(part 1 of 3)
# Autodesk Inventor assembly: COMPONENTS
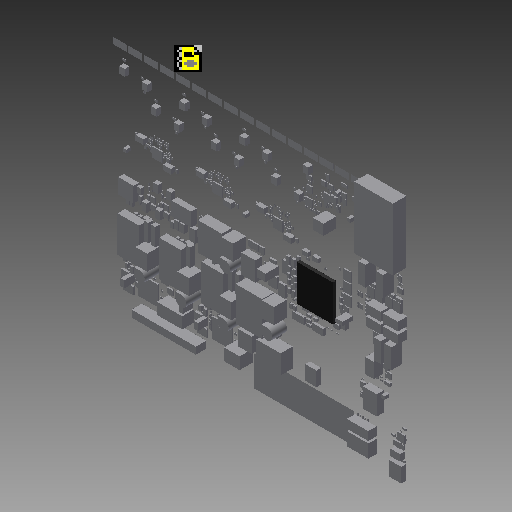
[picture p0: Inventor's stored thumbnail of the model, 512x512]
Saved by Autodesk Inventor 2017 (Build 210142000, 142)
## iProperties
Created: 2016-03-07
Part Number: COMPONENTS
Document SubType Name: Assembly
Designer: rtreacy
Author: rtreacy
## Documents named in this file (794)
- C:\Users\Zara\Documents\hera-cad\Node\SNAP_V2\Workspaces\Workspace\drawings\SNAP Ver2 pack-n-go\Workgroups\NotInProject\COMPONENTS.iam
- C:\Users\Zara\Documents\hera-cad\Node\SNAP_V2\Workspaces\Workspace\drawings\SNAP Ver2 pack-n-go\Workgroups\NotInProject\INDC1005X55L_L30.ipt
- C:\Users\Zara\Documents\hera-cad\Node\SNAP_V2\Workspaces\Workspace\drawings\SNAP Ver2 pack-n-go\Workgroups\NotInProject\INDC1005X55L_L31.ipt
- C:\Users\Zara\Documents\hera-cad\Node\SNAP_V2\Workspaces\Workspace\drawings\SNAP Ver2 pack-n-go\Workgroups\NotInProject\NRAO-LOGO_NOREFDES.ipt
- C:\Users\Zara\Documents\hera-cad\Node\SNAP_V2\Workspaces\Workspace\drawings\SNAP Ver2 pack-n-go\Workgroups\NotInProject\MOLEX_SD-74754-0220_M23.ipt
- C:\Users\Zara\Documents\hera-cad\Node\SNAP_V2\Workspaces\Workspace\drawings\SNAP Ver2 pack-n-go\Workgroups\NotInProject\SHDRRA14W55P200_7X2_1665X100-1_J11.ipt
- C:\Users\Zara\Documents\hera-cad\Node\SNAP_V2\Workspaces\Workspace\drawings\SNAP Ver2 pack-n-go\Workgroups\NotInProject\SHDRV14W55P200_7X2_1665X630H-1_J3.ipt
- C:\Users\Zara\Documents\hera-cad\Node\SNAP_V2\Workspaces\Workspace\drawings\SNAP Ver2 pack-n-go\Workgroups\NotInProject\TE_CONN_6367550-5_P3.ipt
- C:\Users\Zara\Documents\hera-cad\Node\SNAP_V2\Workspaces\Workspace\drawings\SNAP Ver2 pack-n-go\Workgroups\NotInProject\TO170P1430X470-6N-ALT1_U18.ipt
- C:\Users\Zara\Documents\hera-cad\Node\SNAP_V2\Workspaces\Workspace\drawings\SNAP Ver2 pack-n-go\Workgroups\NotInProject\SMA_END_LAUNCH_SMATP1.ipt
- C:\Users\Zara\Documents\hera-cad\Node\SNAP_V2\Workspaces\Workspace\drawings\SNAP Ver2 pack-n-go\Workgroups\NotInProject\SMA_END_LAUNCH_SMATP2.ipt
- C:\Users\Zara\Documents\hera-cad\Node\SNAP_V2\Workspaces\Workspace\drawings\SNAP Ver2 pack-n-go\Workgroups\NotInProject\SMA_END_LAUNCH_SMATP3.ipt
- C:\Users\Zara\Documents\hera-cad\Node\SNAP_V2\Workspaces\Workspace\drawings\SNAP Ver2 pack-n-go\Workgroups\NotInProject\SMA_END_LAUNCH_SMATP4.ipt
- C:\Users\Zara\Documents\hera-cad\Node\SNAP_V2\Workspaces\Workspace\drawings\SNAP Ver2 pack-n-go\Workgroups\NotInProject\SMA_END_LAUNCH_SMATP5.ipt
- C:\Users\Zara\Documents\hera-cad\Node\SNAP_V2\Workspaces\Workspace\drawings\SNAP Ver2 pack-n-go\Workgroups\NotInProject\SMA_END_LAUNCH_SMATP6.ipt
- C:\Users\Zara\Documents\hera-cad\Node\SNAP_V2\Workspaces\Workspace\drawings\SNAP Ver2 pack-n-go\Workgroups\NotInProject\SMA_END_LAUNCH_SMATP7.ipt
- C:\Users\Zara\Documents\hera-cad\Node\SNAP_V2\Workspaces\Workspace\drawings\SNAP Ver2 pack-n-go\Workgroups\NotInProject\SMA_END_LAUNCH_SMATP8.ipt
- C:\Users\Zara\Documents\hera-cad\Node\SNAP_V2\Workspaces\Workspace\drawings\SNAP Ver2 pack-n-go\Workgroups\NotInProject\SMA_END_LAUNCH_SMATP9.ipt
- C:\Users\Zara\Documents\hera-cad\Node\SNAP_V2\Workspaces\Workspace\drawings\SNAP Ver2 pack-n-go\Workgroups\NotInProject\SMA_END_LAUNCH_SMATP10.ipt
- C:\Users\Zara\Documents\hera-cad\Node\SNAP_V2\Workspaces\Workspace\drawings\SNAP Ver2 pack-n-go\Workgroups\NotInProject\SMA_END_LAUNCH_SMATP11.ipt
- C:\Users\Zara\Documents\hera-cad\Node\SNAP_V2\Workspaces\Workspace\drawings\SNAP Ver2 pack-n-go\Workgroups\NotInProject\SMA_END_LAUNCH_SMATP12.ipt
- C:\Users\Zara\Documents\hera-cad\Node\SNAP_V2\Workspaces\Workspace\drawings\SNAP Ver2 pack-n-go\Workgroups\NotInProject\SMA_END_LAUNCH_SMATP13.ipt
- C:\Users\Zara\Documents\hera-cad\Node\SNAP_V2\Workspaces\Workspace\drawings\SNAP Ver2 pack-n-go\Workgroups\NotInProject\SMA_END_LAUNCH_SMATP14.ipt
- C:\Users\Zara\Documents\hera-cad\Node\SNAP_V2\Workspaces\Workspace\drawings\SNAP Ver2 pack-n-go\Workgroups\NotInProject\SMA_END_LAUNCH_SMATP15.ipt
- C:\Users\Zara\Documents\hera-cad\Node\SNAP_V2\Workspaces\Workspace\drawings\SNAP Ver2 pack-n-go\Workgroups\NotInProject\SMA_END_LAUNCH_SMATP16.ipt
- C:\Users\Zara\Documents\hera-cad\Node\SNAP_V2\Workspaces\Workspace\drawings\SNAP Ver2 pack-n-go\Workgroups\NotInProject\HDRV254W64P254R1L508T254H838_JP3.ipt
- C:\Users\Zara\Documents\hera-cad\Node\SNAP_V2\Workspaces\Workspace\drawings\SNAP Ver2 pack-n-go\Workgroups\NotInProject\HDRV254W64P254R1L508T254H838_JP2.ipt
- C:\Users\Zara\Documents\hera-cad\Node\SNAP_V2\Workspaces\Workspace\drawings\SNAP Ver2 pack-n-go\Workgroups\NotInProject\HDRV254W64P254R1L508T254H838_JP1.ipt
- C:\Users\Zara\Documents\hera-cad\Node\SNAP_V2\Workspaces\Workspace\drawings\SNAP Ver2 pack-n-go\Workgroups\NotInProject\HDRV254W64P254R1L508T254H838_JP4.ipt
- C:\Users\Zara\Documents\hera-cad\Node\SNAP_V2\Workspaces\Workspace\drawings\SNAP Ver2 pack-n-go\Workgroups\NotInProject\HDRV6X2_J9.ipt
- C:\Users\Zara\Documents\hera-cad\Node\SNAP_V2\Workspaces\Workspace\drawings\SNAP Ver2 pack-n-go\Workgroups\NotInProject\HDRV6X2_J7.ipt
- C:\Users\Zara\Documents\hera-cad\Node\SNAP_V2\Workspaces\Workspace\drawings\SNAP Ver2 pack-n-go\Workgroups\NotInProject\HDRV6X2_J5.ipt
- C:\Users\Zara\Documents\hera-cad\Node\SNAP_V2\Workspaces\Workspace\drawings\SNAP Ver2 pack-n-go\Workgroups\NotInProject\HDRV6X2_J6.ipt
- C:\Users\Zara\Documents\hera-cad\Node\SNAP_V2\Workspaces\Workspace\drawings\SNAP Ver2 pack-n-go\Workgroups\NotInProject\HDRV2X20_PI2.ipt
- C:\Users\Zara\Documents\hera-cad\Node\SNAP_V2\Workspaces\Workspace\drawings\SNAP Ver2 pack-n-go\Workgroups\NotInProject\CAPPRD350W60D820H1170P_C259.ipt
- C:\Users\Zara\Documents\hera-cad\Node\SNAP_V2\Workspaces\Workspace\drawings\SNAP Ver2 pack-n-go\Workgroups\NotInProject\CAPPRD350W60D820H1170P_C250.ipt
- C:\Users\Zara\Documents\hera-cad\Node\SNAP_V2\Workspaces\Workspace\drawings\SNAP Ver2 pack-n-go\Workgroups\NotInProject\CAPPRD350W60D820H1170P_C241.ipt
- C:\Users\Zara\Documents\hera-cad\Node\SNAP_V2\Workspaces\Workspace\drawings\SNAP Ver2 pack-n-go\Workgroups\NotInProject\CAPPRD350W60D820H1170P_C234.ipt
- C:\Users\Zara\Documents\hera-cad\Node\SNAP_V2\Workspaces\Workspace\drawings\SNAP Ver2 pack-n-go\Workgroups\NotInProject\CAPPRD350W60D820H1170P_C227.ipt
- C:\Users\Zara\Documents\hera-cad\Node\SNAP_V2\Workspaces\Workspace\drawings\SNAP Ver2 pack-n-go\Workgroups\NotInProject\QFN50P500X500X100-28N_U29.ipt
- C:\Users\Zara\Documents\hera-cad\Node\SNAP_V2\Workspaces\Workspace\drawings\SNAP Ver2 pack-n-go\Workgroups\NotInProject\FID100X125_NOREFDES.ipt
- C:\Users\Zara\Documents\hera-cad\Node\SNAP_V2\Workspaces\Workspace\drawings\SNAP Ver2 pack-n-go\Workgroups\NotInProject\DIOAD1365W102L865D350B_D4.ipt
- C:\Users\Zara\Documents\hera-cad\Node\SNAP_V2\Workspaces\Workspace\drawings\SNAP Ver2 pack-n-go\Workgroups\NotInProject\DIOAD1365W102L865D350B_D5.ipt
- C:\Users\Zara\Documents\hera-cad\Node\SNAP_V2\Workspaces\Workspace\drawings\SNAP Ver2 pack-n-go\Workgroups\NotInProject\DIOAD1365W102L865D350B_D6.ipt
- C:\Users\Zara\Documents\hera-cad\Node\SNAP_V2\Workspaces\Workspace\drawings\SNAP Ver2 pack-n-go\Workgroups\NotInProject\DIOAD1365W102L865D350B_D7.ipt
- C:\Users\Zara\Documents\hera-cad\Node\SNAP_V2\Workspaces\Workspace\drawings\SNAP Ver2 pack-n-go\Workgroups\NotInProject\DIOAD1365W102L865D350B_D8.ipt
- C:\Users\Zara\Documents\hera-cad\Node\SNAP_V2\Workspaces\Workspace\drawings\SNAP Ver2 pack-n-go\Workgroups\NotInProject\BGA676C100P26X26_2700X2700X260_U25.ipt
- C:\Users\Zara\Documents\hera-cad\Node\SNAP_V2\Workspaces\Workspace\drawings\SNAP Ver2 pack-n-go\Workgroups\NotInProject\EMERSON_RFCONN_SMA-V_TP2.ipt
- C:\Users\Zara\Documents\hera-cad\Node\SNAP_V2\Workspaces\Workspace\drawings\SNAP Ver2 pack-n-go\Workgroups\NotInProject\FIL_BNX01X_U24.ipt
- C:\Users\Zara\Documents\hera-cad\Node\SNAP_V2\Workspaces\Workspace\drawings\SNAP Ver2 pack-n-go\Workgroups\NotInProject\MOLEX_744410010_P2.ipt
- C:\Users\Zara\Documents\hera-cad\Node\SNAP_V2\Workspaces\Workspace\drawings\SNAP Ver2 pack-n-go\Workgroups\NotInProject\MOLEX_744410010_P1.ipt
- C:\Users\Zara\Documents\hera-cad\Node\SNAP_V2\Workspaces\Workspace\drawings\SNAP Ver2 pack-n-go\Workgroups\NotInProject\SOT89_Q5.ipt
- C:\Users\Zara\Documents\hera-cad\Node\SNAP_V2\Workspaces\Workspace\drawings\SNAP Ver2 pack-n-go\Workgroups\NotInProject\SOT89_Q6.ipt
- C:\Users\Zara\Documents\hera-cad\Node\SNAP_V2\Workspaces\Workspace\drawings\SNAP Ver2 pack-n-go\Workgroups\NotInProject\QFN80P1000X1000X440-42T320X130X2N-ALT1_U20.ipt
- C:\Users\Zara\Documents\hera-cad\Node\SNAP_V2\Workspaces\Workspace\drawings\SNAP Ver2 pack-n-go\Workgroups\NotInProject\HDR_1X2_LOCK_MOLEX_J61.ipt
- C:\Users\Zara\Documents\hera-cad\Node\SNAP_V2\Workspaces\Workspace\drawings\SNAP Ver2 pack-n-go\Workgroups\NotInProject\DIOMELF3514_D14.ipt
- C:\Users\Zara\Documents\hera-cad\Node\SNAP_V2\Workspaces\Workspace\drawings\SNAP Ver2 pack-n-go\Workgroups\NotInProject\SOT230P700X180-4L050N_Q17.ipt
- C:\Users\Zara\Documents\hera-cad\Node\SNAP_V2\Workspaces\Workspace\drawings\SNAP Ver2 pack-n-go\Workgroups\NotInProject\QFP50P1400X1400X100-80N_U40.ipt
- C:\Users\Zara\Documents\hera-cad\Node\SNAP_V2\Workspaces\Workspace\drawings\SNAP Ver2 pack-n-go\Workgroups\NotInProject\QFP50P1400X1400X100-80N_U42.ipt
- C:\Users\Zara\Documents\hera-cad\Node\SNAP_V2\Workspaces\Workspace\drawings\SNAP Ver2 pack-n-go\Workgroups\NotInProject\QFN50P700X700X100-49T540X540L_U7.ipt
- C:\Users\Zara\Documents\hera-cad\Node\SNAP_V2\Workspaces\Workspace\drawings\SNAP Ver2 pack-n-go\Workgroups\NotInProject\QFN50P700X700X100-49T540X540L_U2.ipt
- C:\Users\Zara\Documents\hera-cad\Node\SNAP_V2\Workspaces\Workspace\drawings\SNAP Ver2 pack-n-go\Workgroups\NotInProject\QFN50P700X700X100-49T540X540L_U12.ipt
- C:\Users\Zara\Documents\hera-cad\Node\SNAP_V2\Workspaces\Workspace\drawings\SNAP Ver2 pack-n-go\Workgroups\NotInProject\QFN50P500X500X100-33T320X320L_U21.ipt
- C:\Users\Zara\Documents\hera-cad\Node\SNAP_V2\Workspaces\Workspace\drawings\SNAP Ver2 pack-n-go\Workgroups\NotInProject\QFN50P500X500X100-33T380X380L_U23.ipt
- C:\Users\Zara\Documents\hera-cad\Node\SNAP_V2\Workspaces\Workspace\drawings\SNAP Ver2 pack-n-go\Workgroups\NotInProject\QFN50P400X400X100-25T280X280L_U22.ipt
- C:\Users\Zara\Documents\hera-cad\Node\SNAP_V2\Workspaces\Workspace\drawings\SNAP Ver2 pack-n-go\Workgroups\NotInProject\DCDC-CONV_PTD08D210W-22N_U38.ipt
- C:\Users\Zara\Documents\hera-cad\Node\SNAP_V2\Workspaces\Workspace\drawings\SNAP Ver2 pack-n-go\Workgroups\NotInProject\DCDC-CONV_PTD08D210W-22N_U36.ipt
- C:\Users\Zara\Documents\hera-cad\Node\SNAP_V2\Workspaces\Workspace\drawings\SNAP Ver2 pack-n-go\Workgroups\NotInProject\DCDC-CONV_PTD08D210W-22N_U37.ipt
- C:\Users\Zara\Documents\hera-cad\Node\SNAP_V2\Workspaces\Workspace\drawings\SNAP Ver2 pack-n-go\Workgroups\NotInProject\QFN50P300X300X100-17T178X178L_U17.ipt
- C:\Users\Zara\Documents\hera-cad\Node\SNAP_V2\Workspaces\Workspace\drawings\SNAP Ver2 pack-n-go\Workgroups\NotInProject\QFN50P300X300X100-17T178X178L_U16.ipt
- C:\Users\Zara\Documents\hera-cad\Node\SNAP_V2\Workspaces\Workspace\drawings\SNAP Ver2 pack-n-go\Workgroups\NotInProject\SOP65P640X120-16N_U41.ipt
- C:\Users\Zara\Documents\hera-cad\Node\SNAP_V2\Workspaces\Workspace\drawings\SNAP Ver2 pack-n-go\Workgroups\NotInProject\SOP65P640X120-16N_U39.ipt
- C:\Users\Zara\Documents\hera-cad\Node\SNAP_V2\Workspaces\Workspace\drawings\SNAP Ver2 pack-n-go\Workgroups\NotInProject\QFN40P260X180X55-16L_U28.ipt
- C:\Users\Zara\Documents\hera-cad\Node\SNAP_V2\Workspaces\Workspace\drawings\SNAP Ver2 pack-n-go\Workgroups\NotInProject\QFN40P260X180X55-16L_U46.ipt
- C:\Users\Zara\Documents\hera-cad\Node\SNAP_V2\Workspaces\Workspace\drawings\SNAP Ver2 pack-n-go\Workgroups\NotInProject\QFN40P260X180X55-16L_U47.ipt
- C:\Users\Zara\Documents\hera-cad\Node\SNAP_V2\Workspaces\Workspace\drawings\SNAP Ver2 pack-n-go\Workgroups\NotInProject\DCDC-CONV_PTD08A020WAD-12N_U35.ipt
- C:\Users\Zara\Documents\hera-cad\Node\SNAP_V2\Workspaces\Workspace\drawings\SNAP Ver2 pack-n-go\Workgroups\NotInProject\DCDC-CONV_PTD08A010WAD-12N_U34.ipt
- C:\Users\Zara\Documents\hera-cad\Node\SNAP_V2\Workspaces\Workspace\drawings\SNAP Ver2 pack-n-go\Workgroups\NotInProject\HDRV1016W64P254R2L2032T905H900_J1.ipt
- C:\Users\Zara\Documents\hera-cad\Node\SNAP_V2\Workspaces\Workspace\drawings\SNAP Ver2 pack-n-go\Workgroups\NotInProject\SW_SDA05H1SBD_S2.ipt
- C:\Users\Zara\Documents\hera-cad\Node\SNAP_V2\Workspaces\Workspace\drawings\SNAP Ver2 pack-n-go\Workgroups\NotInProject\SW_SDA05H1SBD_S1.ipt
- C:\Users\Zara\Documents\hera-cad\Node\SNAP_V2\Workspaces\Workspace\drawings\SNAP Ver2 pack-n-go\Workgroups\NotInProject\MOLEX_548190589_J4.ipt
- C:\Users\Zara\Documents\hera-cad\Node\SNAP_V2\Workspaces\Workspace\drawings\SNAP Ver2 pack-n-go\Workgroups\NotInProject\SOP50P310X90-8N_U44.ipt
- C:\Users\Zara\Documents\hera-cad\Node\SNAP_V2\Workspaces\Workspace\drawings\SNAP Ver2 pack-n-go\Workgroups\NotInProject\SOP50P310X90-8N_U45.ipt
- C:\Users\Zara\Documents\hera-cad\Node\SNAP_V2\Workspaces\Workspace\drawings\SNAP Ver2 pack-n-go\Workgroups\NotInProject\OSC254P700X500X90-7T147X230N_U32.ipt
- C:\Users\Zara\Documents\hera-cad\Node\SNAP_V2\Workspaces\Workspace\drawings\SNAP Ver2 pack-n-go\Workgroups\NotInProject\MOLEX_39301060_J2.ipt
- C:\Users\Zara\Documents\hera-cad\Node\SNAP_V2\Workspaces\Workspace\drawings\SNAP Ver2 pack-n-go\Workgroups\NotInProject\SOT95P280X145-6N_U26.ipt
- C:\Users\Zara\Documents\hera-cad\Node\SNAP_V2\Workspaces\Workspace\drawings\SNAP Ver2 pack-n-go\Workgroups\NotInProject\OSC254P700X500X90-6N_U48.ipt
- C:\Users\Zara\Documents\hera-cad\Node\SNAP_V2\Workspaces\Workspace\drawings\SNAP Ver2 pack-n-go\Workgroups\NotInProject\OSC254P700X500X90-6N_U33.ipt
- C:\Users\Zara\Documents\hera-cad\Node\SNAP_V2\Workspaces\Workspace\drawings\SNAP Ver2 pack-n-go\Workgroups\NotInProject\XFMR_TC1-1-13MG2_T11.ipt
- C:\Users\Zara\Documents\hera-cad\Node\SNAP_V2\Workspaces\Workspace\drawings\SNAP Ver2 pack-n-go\Workgroups\NotInProject\XFMR_TC1-1-13MG2_T10.ipt
- C:\Users\Zara\Documents\hera-cad\Node\SNAP_V2\Workspaces\Workspace\drawings\SNAP Ver2 pack-n-go\Workgroups\NotInProject\XFMR_TC1-1-13MG2_T4.ipt
- C:\Users\Zara\Documents\hera-cad\Node\SNAP_V2\Workspaces\Workspace\drawings\SNAP Ver2 pack-n-go\Workgroups\NotInProject\XFMR_TC1-1-13MG2_T6.ipt
- C:\Users\Zara\Documents\hera-cad\Node\SNAP_V2\Workspaces\Workspace\drawings\SNAP Ver2 pack-n-go\Workgroups\NotInProject\XFMR_TC1-1-13MG2_T12.ipt
- C:\Users\Zara\Documents\hera-cad\Node\SNAP_V2\Workspaces\Workspace\drawings\SNAP Ver2 pack-n-go\Workgroups\NotInProject\XFMR_TC1-1-13MG2_T5.ipt
- C:\Users\Zara\Documents\hera-cad\Node\SNAP_V2\Workspaces\Workspace\drawings\SNAP Ver2 pack-n-go\Workgroups\NotInProject\XFMR_TC1-1-13MG2_T3.ipt
- C:\Users\Zara\Documents\hera-cad\Node\SNAP_V2\Workspaces\Workspace\drawings\SNAP Ver2 pack-n-go\Workgroups\NotInProject\XFMR_TC1-1-13MG2_T8.ipt
- C:\Users\Zara\Documents\hera-cad\Node\SNAP_V2\Workspaces\Workspace\drawings\SNAP Ver2 pack-n-go\Workgroups\NotInProject\XFMR_TC1-1-13MG2_T9.ipt
- C:\Users\Zara\Documents\hera-cad\Node\SNAP_V2\Workspaces\Workspace\drawings\SNAP Ver2 pack-n-go\Workgroups\NotInProject\XFMR_TC1-1-13MG2_T13.ipt
- C:\Users\Zara\Documents\hera-cad\Node\SNAP_V2\Workspaces\Workspace\drawings\SNAP Ver2 pack-n-go\Workgroups\NotInProject\XFMR_TC1-1-13MG2_T2.ipt
- C:\Users\Zara\Documents\hera-cad\Node\SNAP_V2\Workspaces\Workspace\drawings\SNAP Ver2 pack-n-go\Workgroups\NotInProject\XFMR_TC1-1-13MG2_T7.ipt
- C:\Users\Zara\Documents\hera-cad\Node\SNAP_V2\Workspaces\Workspace\drawings\SNAP Ver2 pack-n-go\Workgroups\NotInProject\XFMR_TC1-1-13MG2_T1.ipt
- C:\Users\Zara\Documents\hera-cad\Node\SNAP_V2\Workspaces\Workspace\drawings\SNAP Ver2 pack-n-go\Workgroups\NotInProject\SOT95P280X145-5N_U30.ipt
- C:\Users\Zara\Documents\hera-cad\Node\SNAP_V2\Workspaces\Workspace\drawings\SNAP Ver2 pack-n-go\Workgroups\NotInProject\SOT95P280X145-5N_U19.ipt
- C:\Users\Zara\Documents\hera-cad\Node\SNAP_V2\Workspaces\Workspace\drawings\SNAP Ver2 pack-n-go\Workgroups\NotInProject\SOT143R_X1.ipt
- C:\Users\Zara\Documents\hera-cad\Node\SNAP_V2\Workspaces\Workspace\drawings\SNAP Ver2 pack-n-go\Workgroups\NotInProject\RESCAF65P100X100X45-4N_U10.ipt
- C:\Users\Zara\Documents\hera-cad\Node\SNAP_V2\Workspaces\Workspace\drawings\SNAP Ver2 pack-n-go\Workgroups\NotInProject\RESCAF65P100X100X45-4N_U1.ipt
- C:\Users\Zara\Documents\hera-cad\Node\SNAP_V2\Workspaces\Workspace\drawings\SNAP Ver2 pack-n-go\Workgroups\NotInProject\RESCAF65P100X100X45-4N_U11.ipt
- C:\Users\Zara\Documents\hera-cad\Node\SNAP_V2\Workspaces\Workspace\drawings\SNAP Ver2 pack-n-go\Workgroups\NotInProject\RESCAF65P100X100X45-4N_U13.ipt
- C:\Users\Zara\Documents\hera-cad\Node\SNAP_V2\Workspaces\Workspace\drawings\SNAP Ver2 pack-n-go\Workgroups\NotInProject\RESCAF65P100X100X45-4N_U14.ipt
- C:\Users\Zara\Documents\hera-cad\Node\SNAP_V2\Workspaces\Workspace\drawings\SNAP Ver2 pack-n-go\Workgroups\NotInProject\RESCAF65P100X100X45-4N_U15.ipt
- C:\Users\Zara\Documents\hera-cad\Node\SNAP_V2\Workspaces\Workspace\drawings\SNAP Ver2 pack-n-go\Workgroups\NotInProject\RESCAF65P100X100X45-4N_U3.ipt
- C:\Users\Zara\Documents\hera-cad\Node\SNAP_V2\Workspaces\Workspace\drawings\SNAP Ver2 pack-n-go\Workgroups\NotInProject\RESCAF65P100X100X45-4N_U4.ipt
- C:\Users\Zara\Documents\hera-cad\Node\SNAP_V2\Workspaces\Workspace\drawings\SNAP Ver2 pack-n-go\Workgroups\NotInProject\RESCAF65P100X100X45-4N_U5.ipt
- C:\Users\Zara\Documents\hera-cad\Node\SNAP_V2\Workspaces\Workspace\drawings\SNAP Ver2 pack-n-go\Workgroups\NotInProject\RESCAF65P100X100X45-4N_U6.ipt
- C:\Users\Zara\Documents\hera-cad\Node\SNAP_V2\Workspaces\Workspace\drawings\SNAP Ver2 pack-n-go\Workgroups\NotInProject\RESCAF65P100X100X45-4N_U8.ipt
- C:\Users\Zara\Documents\hera-cad\Node\SNAP_V2\Workspaces\Workspace\drawings\SNAP Ver2 pack-n-go\Workgroups\NotInProject\RESCAF65P100X100X45-4N_U9.ipt
- C:\Users\Zara\Documents\hera-cad\Node\SNAP_V2\Workspaces\Workspace\drawings\SNAP Ver2 pack-n-go\Workgroups\NotInProject\SW_TL3301EF100QG_SW5.ipt
- C:\Users\Zara\Documents\hera-cad\Node\SNAP_V2\Workspaces\Workspace\drawings\SNAP Ver2 pack-n-go\Workgroups\NotInProject\SW_TL3301EF100QG_SW4.ipt
- C:\Users\Zara\Documents\hera-cad\Node\SNAP_V2\Workspaces\Workspace\drawings\SNAP Ver2 pack-n-go\Workgroups\NotInProject\SW_TL3301EF100QG_SW3.ipt
- C:\Users\Zara\Documents\hera-cad\Node\SNAP_V2\Workspaces\Workspace\drawings\SNAP Ver2 pack-n-go\Workgroups\NotInProject\SW_TL3301EF100QG_SW2.ipt
- C:\Users\Zara\Documents\hera-cad\Node\SNAP_V2\Workspaces\Workspace\drawings\SNAP Ver2 pack-n-go\Workgroups\NotInProject\SW_TL3301EF100QG_SW1.ipt
- C:\Users\Zara\Documents\hera-cad\Node\SNAP_V2\Workspaces\Workspace\drawings\SNAP Ver2 pack-n-go\Workgroups\NotInProject\SOT192P237X112-4L20N_D3.ipt
- C:\Users\Zara\Documents\hera-cad\Node\SNAP_V2\Workspaces\Workspace\drawings\SNAP Ver2 pack-n-go\Workgroups\NotInProject\SOT95P237X100-4_Q1.ipt
- C:\Users\Zara\Documents\hera-cad\Node\SNAP_V2\Workspaces\Workspace\drawings\SNAP Ver2 pack-n-go\Workgroups\NotInProject\SOT95P237X100-4_Q4.ipt
- C:\Users\Zara\Documents\hera-cad\Node\SNAP_V2\Workspaces\Workspace\drawings\SNAP Ver2 pack-n-go\Workgroups\NotInProject\SOT95P237X100-4_Q3.ipt
- C:\Users\Zara\Documents\hera-cad\Node\SNAP_V2\Workspaces\Workspace\drawings\SNAP Ver2 pack-n-go\Workgroups\NotInProject\SOT95P237X100-4_Q2.ipt
- C:\Users\Zara\Documents\hera-cad\Node\SNAP_V2\Workspaces\Workspace\drawings\SNAP Ver2 pack-n-go\Workgroups\NotInProject\SOT95P237X100-4_Q8.ipt
- C:\Users\Zara\Documents\hera-cad\Node\SNAP_V2\Workspaces\Workspace\drawings\SNAP Ver2 pack-n-go\Workgroups\NotInProject\SOT95P237X100-4_Q7.ipt
- C:\Users\Zara\Documents\hera-cad\Node\SNAP_V2\Workspaces\Workspace\drawings\SNAP Ver2 pack-n-go\Workgroups\NotInProject\SOT95P240X110-3L16N_U31.ipt
- C:\Users\Zara\Documents\hera-cad\Node\SNAP_V2\Workspaces\Workspace\drawings\SNAP Ver2 pack-n-go\Workgroups\NotInProject\SOT95P240X110-3L16N_D1.ipt
- C:\Users\Zara\Documents\hera-cad\Node\SNAP_V2\Workspaces\Workspace\drawings\SNAP Ver2 pack-n-go\Workgroups\NotInProject\SOT95P240X110-3L16N_D2.ipt
- C:\Users\Zara\Documents\hera-cad\Node\SNAP_V2\Workspaces\Workspace\drawings\SNAP Ver2 pack-n-go\Workgroups\NotInProject\CAPC1005X50L_C604.ipt
- C:\Users\Zara\Documents\hera-cad\Node\SNAP_V2\Workspaces\Workspace\drawings\SNAP Ver2 pack-n-go\Workgroups\NotInProject\CAPC1005X50L_C603.ipt
- C:\Users\Zara\Documents\hera-cad\Node\SNAP_V2\Workspaces\Workspace\drawings\SNAP Ver2 pack-n-go\Workgroups\NotInProject\CAPC1005X50L_C591.ipt
- C:\Users\Zara\Documents\hera-cad\Node\SNAP_V2\Workspaces\Workspace\drawings\SNAP Ver2 pack-n-go\Workgroups\NotInProject\CAPC1005X50L_C592.ipt
- C:\Users\Zara\Documents\hera-cad\Node\SNAP_V2\Workspaces\Workspace\drawings\SNAP Ver2 pack-n-go\Workgroups\NotInProject\CAPC1005X50L_C593.ipt
- C:\Users\Zara\Documents\hera-cad\Node\SNAP_V2\Workspaces\Workspace\drawings\SNAP Ver2 pack-n-go\Workgroups\NotInProject\CAPC1005X50L_C46.ipt
- C:\Users\Zara\Documents\hera-cad\Node\SNAP_V2\Workspaces\Workspace\drawings\SNAP Ver2 pack-n-go\Workgroups\NotInProject\CAPC1005X50L_C51.ipt
- C:\Users\Zara\Documents\hera-cad\Node\SNAP_V2\Workspaces\Workspace\drawings\SNAP Ver2 pack-n-go\Workgroups\NotInProject\CAPC1005X50L_C57.ipt
- C:\Users\Zara\Documents\hera-cad\Node\SNAP_V2\Workspaces\Workspace\drawings\SNAP Ver2 pack-n-go\Workgroups\NotInProject\CAPC1005X50L_C7.ipt
- C:\Users\Zara\Documents\hera-cad\Node\SNAP_V2\Workspaces\Workspace\drawings\SNAP Ver2 pack-n-go\Workgroups\NotInProject\CAPC1005X50L_C82.ipt
- C:\Users\Zara\Documents\hera-cad\Node\SNAP_V2\Workspaces\Workspace\drawings\SNAP Ver2 pack-n-go\Workgroups\NotInProject\CAPC1005X50L_C43.ipt
- C:\Users\Zara\Documents\hera-cad\Node\SNAP_V2\Workspaces\Workspace\drawings\SNAP Ver2 pack-n-go\Workgroups\NotInProject\CAPC1005X50L_C96.ipt
- C:\Users\Zara\Documents\hera-cad\Node\SNAP_V2\Workspaces\Workspace\drawings\SNAP Ver2 pack-n-go\Workgroups\NotInProject\CAPC1005X50L_C85.ipt
- C:\Users\Zara\Documents\hera-cad\Node\SNAP_V2\Workspaces\Workspace\drawings\SNAP Ver2 pack-n-go\Workgroups\NotInProject\CAPC1005X50L_C90.ipt
- C:\Users\Zara\Documents\hera-cad\Node\SNAP_V2\Workspaces\Workspace\drawings\SNAP Ver2 pack-n-go\Workgroups\NotInProject\CAPC1005X50L_C13.ipt
- C:\Users\Zara\Documents\hera-cad\Node\SNAP_V2\Workspaces\Workspace\drawings\SNAP Ver2 pack-n-go\Workgroups\NotInProject\CAPC1005X50L_C4.ipt
- C:\Users\Zara\Documents\hera-cad\Node\SNAP_V2\Workspaces\Workspace\drawings\SNAP Ver2 pack-n-go\Workgroups\NotInProject\CAPC1005X50L_C47.ipt
- C:\Users\Zara\Documents\hera-cad\Node\SNAP_V2\Workspaces\Workspace\drawings\SNAP Ver2 pack-n-go\Workgroups\NotInProject\CAPC1005X50L_C5.ipt
- C:\Users\Zara\Documents\hera-cad\Node\SNAP_V2\Workspaces\Workspace\drawings\SNAP Ver2 pack-n-go\Workgroups\NotInProject\CAPC1005X50L_C52.ipt
- C:\Users\Zara\Documents\hera-cad\Node\SNAP_V2\Workspaces\Workspace\drawings\SNAP Ver2 pack-n-go\Workgroups\NotInProject\CAPC1005X50L_C58.ipt
- C:\Users\Zara\Documents\hera-cad\Node\SNAP_V2\Workspaces\Workspace\drawings\SNAP Ver2 pack-n-go\Workgroups\NotInProject\CAPC1005X50L_C8.ipt
- C:\Users\Zara\Documents\hera-cad\Node\SNAP_V2\Workspaces\Workspace\drawings\SNAP Ver2 pack-n-go\Workgroups\NotInProject\CAPC1005X50L_C83.ipt
- C:\Users\Zara\Documents\hera-cad\Node\SNAP_V2\Workspaces\Workspace\drawings\SNAP Ver2 pack-n-go\Workgroups\NotInProject\CAPC1005X50L_C86.ipt
- C:\Users\Zara\Documents\hera-cad\Node\SNAP_V2\Workspaces\Workspace\drawings\SNAP Ver2 pack-n-go\Workgroups\NotInProject\CAPC1005X50L_C91.ipt
- C:\Users\Zara\Documents\hera-cad\Node\SNAP_V2\Workspaces\Workspace\drawings\SNAP Ver2 pack-n-go\Workgroups\NotInProject\CAPC1005X50L_C97.ipt
- C:\Users\Zara\Documents\hera-cad\Node\SNAP_V2\Workspaces\Workspace\drawings\SNAP Ver2 pack-n-go\Workgroups\NotInProject\CAPC1005X50L_C19.ipt
- C:\Users\Zara\Documents\hera-cad\Node\SNAP_V2\Workspaces\Workspace\drawings\SNAP Ver2 pack-n-go\Workgroups\NotInProject\CAPC1005X50L_C14.ipt
- C:\Users\Zara\Documents\hera-cad\Node\SNAP_V2\Workspaces\Workspace\drawings\SNAP Ver2 pack-n-go\Workgroups\NotInProject\CAPC1005X50L_C17.ipt
- C:\Users\Zara\Documents\hera-cad\Node\SNAP_V2\Workspaces\Workspace\drawings\SNAP Ver2 pack-n-go\Workgroups\NotInProject\CAPC1005X50L_C2.ipt
- C:\Users\Zara\Documents\hera-cad\Node\SNAP_V2\Workspaces\Workspace\drawings\SNAP Ver2 pack-n-go\Workgroups\NotInProject\CAPC1005X50L_C41.ipt
- C:\Users\Zara\Documents\hera-cad\Node\SNAP_V2\Workspaces\Workspace\drawings\SNAP Ver2 pack-n-go\Workgroups\NotInProject\CAPC1005X50L_C44.ipt
- C:\Users\Zara\Documents\hera-cad\Node\SNAP_V2\Workspaces\Workspace\drawings\SNAP Ver2 pack-n-go\Workgroups\NotInProject\CAPC1005X50L_C53.ipt
- C:\Users\Zara\Documents\hera-cad\Node\SNAP_V2\Workspaces\Workspace\drawings\SNAP Ver2 pack-n-go\Workgroups\NotInProject\CAPC1005X50L_C80.ipt
- C:\Users\Zara\Documents\hera-cad\Node\SNAP_V2\Workspaces\Workspace\drawings\SNAP Ver2 pack-n-go\Workgroups\NotInProject\CAPC1005X50L_C87.ipt
- C:\Users\Zara\Documents\hera-cad\Node\SNAP_V2\Workspaces\Workspace\drawings\SNAP Ver2 pack-n-go\Workgroups\NotInProject\CAPC1005X50L_C9.ipt
- C:\Users\Zara\Documents\hera-cad\Node\SNAP_V2\Workspaces\Workspace\drawings\SNAP Ver2 pack-n-go\Workgroups\NotInProject\CAPC1005X50L_C92.ipt
- C:\Users\Zara\Documents\hera-cad\Node\SNAP_V2\Workspaces\Workspace\drawings\SNAP Ver2 pack-n-go\Workgroups\NotInProject\CAPC1005X50L_C95.ipt
- C:\Users\Zara\Documents\hera-cad\Node\SNAP_V2\Workspaces\Workspace\drawings\SNAP Ver2 pack-n-go\Workgroups\NotInProject\CAPC1005X50L_C48.ipt
- C:\Users\Zara\Documents\hera-cad\Node\SNAP_V2\Workspaces\Workspace\drawings\SNAP Ver2 pack-n-go\Workgroups\NotInProject\CAPC1005X50L_C148.ipt
- C:\Users\Zara\Documents\hera-cad\Node\SNAP_V2\Workspaces\Workspace\drawings\SNAP Ver2 pack-n-go\Workgroups\NotInProject\CAPC1005X50L_C56.ipt
- C:\Users\Zara\Documents\hera-cad\Node\SNAP_V2\Workspaces\Workspace\drawings\SNAP Ver2 pack-n-go\Workgroups\NotInProject\CAPC1005X50L_C194.ipt
- C:\Users\Zara\Documents\hera-cad\Node\SNAP_V2\Workspaces\Workspace\drawings\SNAP Ver2 pack-n-go\Workgroups\NotInProject\CAPC1005X50L_C195.ipt
- C:\Users\Zara\Documents\hera-cad\Node\SNAP_V2\Workspaces\Workspace\drawings\SNAP Ver2 pack-n-go\Workgroups\NotInProject\CAPC1005X50L_C217.ipt
- C:\Users\Zara\Documents\hera-cad\Node\SNAP_V2\Workspaces\Workspace\drawings\SNAP Ver2 pack-n-go\Workgroups\NotInProject\CAPC1005X50L_C219.ipt
- C:\Users\Zara\Documents\hera-cad\Node\SNAP_V2\Workspaces\Workspace\drawings\SNAP Ver2 pack-n-go\Workgroups\NotInProject\CAPC1005X50L_C220.ipt
- C:\Users\Zara\Documents\hera-cad\Node\SNAP_V2\Workspaces\Workspace\drawings\SNAP Ver2 pack-n-go\Workgroups\NotInProject\CAPC1005X50L_C222.ipt
- C:\Users\Zara\Documents\hera-cad\Node\SNAP_V2\Workspaces\Workspace\drawings\SNAP Ver2 pack-n-go\Workgroups\NotInProject\CAPC1005X50L_C223.ipt
- C:\Users\Zara\Documents\hera-cad\Node\SNAP_V2\Workspaces\Workspace\drawings\SNAP Ver2 pack-n-go\Workgroups\NotInProject\CAPC1005X50L_C224.ipt
- C:\Users\Zara\Documents\hera-cad\Node\SNAP_V2\Workspaces\Workspace\drawings\SNAP Ver2 pack-n-go\Workgroups\NotInProject\CAPC1005X50L_C225.ipt
- C:\Users\Zara\Documents\hera-cad\Node\SNAP_V2\Workspaces\Workspace\drawings\SNAP Ver2 pack-n-go\Workgroups\NotInProject\CAPC1005X50L_C226.ipt
- C:\Users\Zara\Documents\hera-cad\Node\SNAP_V2\Workspaces\Workspace\drawings\SNAP Ver2 pack-n-go\Workgroups\NotInProject\CAPC1005X50L_C269.ipt
- C:\Users\Zara\Documents\hera-cad\Node\SNAP_V2\Workspaces\Workspace\drawings\SNAP Ver2 pack-n-go\Workgroups\NotInProject\CAPC1005X50L_C270.ipt
- C:\Users\Zara\Documents\hera-cad\Node\SNAP_V2\Workspaces\Workspace\drawings\SNAP Ver2 pack-n-go\Workgroups\NotInProject\CAPC1005X50L_C271.ipt
- C:\Users\Zara\Documents\hera-cad\Node\SNAP_V2\Workspaces\Workspace\drawings\SNAP Ver2 pack-n-go\Workgroups\NotInProject\CAPC1005X50L_C273.ipt
- C:\Users\Zara\Documents\hera-cad\Node\SNAP_V2\Workspaces\Workspace\drawings\SNAP Ver2 pack-n-go\Workgroups\NotInProject\CAPC1005X50L_C275.ipt
- C:\Users\Zara\Documents\hera-cad\Node\SNAP_V2\Workspaces\Workspace\drawings\SNAP Ver2 pack-n-go\Workgroups\NotInProject\CAPC1005X50L_C276.ipt
- C:\Users\Zara\Documents\hera-cad\Node\SNAP_V2\Workspaces\Workspace\drawings\SNAP Ver2 pack-n-go\Workgroups\NotInProject\CAPC1005X50L_C277.ipt
- C:\Users\Zara\Documents\hera-cad\Node\SNAP_V2\Workspaces\Workspace\drawings\SNAP Ver2 pack-n-go\Workgroups\NotInProject\CAPC1005X50L_C285.ipt
- C:\Users\Zara\Documents\hera-cad\Node\SNAP_V2\Workspaces\Workspace\drawings\SNAP Ver2 pack-n-go\Workgroups\NotInProject\CAPC1005X50L_C286.ipt
- C:\Users\Zara\Documents\hera-cad\Node\SNAP_V2\Workspaces\Workspace\drawings\SNAP Ver2 pack-n-go\Workgroups\NotInProject\CAPC1005X50L_C291.ipt
- C:\Users\Zara\Documents\hera-cad\Node\SNAP_V2\Workspaces\Workspace\drawings\SNAP Ver2 pack-n-go\Workgroups\NotInProject\CAPC1005X50L_C292.ipt
- C:\Users\Zara\Documents\hera-cad\Node\SNAP_V2\Workspaces\Workspace\drawings\SNAP Ver2 pack-n-go\Workgroups\NotInProject\CAPC1005X50L_C293.ipt
- C:\Users\Zara\Documents\hera-cad\Node\SNAP_V2\Workspaces\Workspace\drawings\SNAP Ver2 pack-n-go\Workgroups\NotInProject\CAPC1005X50L_C295.ipt
- C:\Users\Zara\Documents\hera-cad\Node\SNAP_V2\Workspaces\Workspace\drawings\SNAP Ver2 pack-n-go\Workgroups\NotInProject\CAPC1005X50L_C297.ipt
- C:\Users\Zara\Documents\hera-cad\Node\SNAP_V2\Workspaces\Workspace\drawings\SNAP Ver2 pack-n-go\Workgroups\NotInProject\CAPC1005X50L_C298.ipt
- C:\Users\Zara\Documents\hera-cad\Node\SNAP_V2\Workspaces\Workspace\drawings\SNAP Ver2 pack-n-go\Workgroups\NotInProject\CAPC1005X50L_C299.ipt
- C:\Users\Zara\Documents\hera-cad\Node\SNAP_V2\Workspaces\Workspace\drawings\SNAP Ver2 pack-n-go\Workgroups\NotInProject\CAPC1005X50L_C307.ipt
- C:\Users\Zara\Documents\hera-cad\Node\SNAP_V2\Workspaces\Workspace\drawings\SNAP Ver2 pack-n-go\Workgroups\NotInProject\CAPC1005X50L_C308.ipt
- C:\Users\Zara\Documents\hera-cad\Node\SNAP_V2\Workspaces\Workspace\drawings\SNAP Ver2 pack-n-go\Workgroups\NotInProject\CAPC1005X50L_C312.ipt
- C:\Users\Zara\Documents\hera-cad\Node\SNAP_V2\Workspaces\Workspace\drawings\SNAP Ver2 pack-n-go\Workgroups\NotInProject\CAPC1005X50L_C313.ipt
- C:\Users\Zara\Documents\hera-cad\Node\SNAP_V2\Workspaces\Workspace\drawings\SNAP Ver2 pack-n-go\Workgroups\NotInProject\CAPC1005X50L_C315.ipt
- C:\Users\Zara\Documents\hera-cad\Node\SNAP_V2\Workspaces\Workspace\drawings\SNAP Ver2 pack-n-go\Workgroups\NotInProject\CAPC1005X50L_C317.ipt
- C:\Users\Zara\Documents\hera-cad\Node\SNAP_V2\Workspaces\Workspace\drawings\SNAP Ver2 pack-n-go\Workgroups\NotInProject\CAPC1005X50L_C318.ipt
- C:\Users\Zara\Documents\hera-cad\Node\SNAP_V2\Workspaces\Workspace\drawings\SNAP Ver2 pack-n-go\Workgroups\NotInProject\CAPC1005X50L_C319.ipt
- C:\Users\Zara\Documents\hera-cad\Node\SNAP_V2\Workspaces\Workspace\drawings\SNAP Ver2 pack-n-go\Workgroups\NotInProject\CAPC1005X50L_C321.ipt
- C:\Users\Zara\Documents\hera-cad\Node\SNAP_V2\Workspaces\Workspace\drawings\SNAP Ver2 pack-n-go\Workgroups\NotInProject\CAPC1005X50L_C323.ipt
- C:\Users\Zara\Documents\hera-cad\Node\SNAP_V2\Workspaces\Workspace\drawings\SNAP Ver2 pack-n-go\Workgroups\NotInProject\CAPC1005X50L_C324.ipt
- C:\Users\Zara\Documents\hera-cad\Node\SNAP_V2\Workspaces\Workspace\drawings\SNAP Ver2 pack-n-go\Workgroups\NotInProject\CAPC1005X50L_C325.ipt
- C:\Users\Zara\Documents\hera-cad\Node\SNAP_V2\Workspaces\Workspace\drawings\SNAP Ver2 pack-n-go\Workgroups\NotInProject\CAPC1005X50L_C326.ipt
- C:\Users\Zara\Documents\hera-cad\Node\SNAP_V2\Workspaces\Workspace\drawings\SNAP Ver2 pack-n-go\Workgroups\NotInProject\CAPC1005X50L_C327.ipt
- C:\Users\Zara\Documents\hera-cad\Node\SNAP_V2\Workspaces\Workspace\drawings\SNAP Ver2 pack-n-go\Workgroups\NotInProject\CAPC1005X50L_C328.ipt
- C:\Users\Zara\Documents\hera-cad\Node\SNAP_V2\Workspaces\Workspace\drawings\SNAP Ver2 pack-n-go\Workgroups\NotInProject\CAPC1005X50L_C15.ipt
- C:\Users\Zara\Documents\hera-cad\Node\SNAP_V2\Workspaces\Workspace\drawings\SNAP Ver2 pack-n-go\Workgroups\NotInProject\CAPC1005X50L_C54.ipt
- C:\Users\Zara\Documents\hera-cad\Node\SNAP_V2\Workspaces\Workspace\drawings\SNAP Ver2 pack-n-go\Workgroups\NotInProject\CAPC1005X50L_C192.ipt
- C:\Users\Zara\Documents\hera-cad\Node\SNAP_V2\Workspaces\Workspace\drawings\SNAP Ver2 pack-n-go\Workgroups\NotInProject\CAPC1005X50L_C151.ipt
- C:\Users\Zara\Documents\hera-cad\Node\SNAP_V2\Workspaces\Workspace\drawings\SNAP Ver2 pack-n-go\Workgroups\NotInProject\CAPC1005X50L_C152.ipt
- C:\Users\Zara\Documents\hera-cad\Node\SNAP_V2\Workspaces\Workspace\drawings\SNAP Ver2 pack-n-go\Workgroups\NotInProject\CAPC1005X50L_C153.ipt
- C:\Users\Zara\Documents\hera-cad\Node\SNAP_V2\Workspaces\Workspace\drawings\SNAP Ver2 pack-n-go\Workgroups\NotInProject\CAPC1005X50L_C154.ipt
- C:\Users\Zara\Documents\hera-cad\Node\SNAP_V2\Workspaces\Workspace\drawings\SNAP Ver2 pack-n-go\Workgroups\NotInProject\CAPC1005X50L_C157.ipt
- C:\Users\Zara\Documents\hera-cad\Node\SNAP_V2\Workspaces\Workspace\drawings\SNAP Ver2 pack-n-go\Workgroups\NotInProject\CAPC1005X50L_C160.ipt
- C:\Users\Zara\Documents\hera-cad\Node\SNAP_V2\Workspaces\Workspace\drawings\SNAP Ver2 pack-n-go\Workgroups\NotInProject\CAPC1005X50L_C164.ipt
- C:\Users\Zara\Documents\hera-cad\Node\SNAP_V2\Workspaces\Workspace\drawings\SNAP Ver2 pack-n-go\Workgroups\NotInProject\CAPC1005X50L_C167.ipt
- C:\Users\Zara\Documents\hera-cad\Node\SNAP_V2\Workspaces\Workspace\drawings\SNAP Ver2 pack-n-go\Workgroups\NotInProject\CAPC1005X50L_C172.ipt
- C:\Users\Zara\Documents\hera-cad\Node\SNAP_V2\Workspaces\Workspace\drawings\SNAP Ver2 pack-n-go\Workgroups\NotInProject\CAPC1005X50L_C176.ipt
- C:\Users\Zara\Documents\hera-cad\Node\SNAP_V2\Workspaces\Workspace\drawings\SNAP Ver2 pack-n-go\Workgroups\NotInProject\CAPC1005X50L_C178.ipt
- C:\Users\Zara\Documents\hera-cad\Node\SNAP_V2\Workspaces\Workspace\drawings\SNAP Ver2 pack-n-go\Workgroups\NotInProject\CAPC1005X50L_C16.ipt
- C:\Users\Zara\Documents\hera-cad\Node\SNAP_V2\Workspaces\Workspace\drawings\SNAP Ver2 pack-n-go\Workgroups\NotInProject\CAPC1005X50L_C55.ipt
- C:\Users\Zara\Documents\hera-cad\Node\SNAP_V2\Workspaces\Workspace\drawings\SNAP Ver2 pack-n-go\Workgroups\NotInProject\CAPC1005X50L_C94.ipt
- C:\Users\Zara\Documents\hera-cad\Node\SNAP_V2\Workspaces\Workspace\drawings\SNAP Ver2 pack-n-go\Workgroups\NotInProject\CAPC1005X50L_C168.ipt
- C:\Users\Zara\Documents\hera-cad\Node\SNAP_V2\Workspaces\Workspace\drawings\SNAP Ver2 pack-n-go\Workgroups\NotInProject\CAPC1005X50L_C173.ipt
- C:\Users\Zara\Documents\hera-cad\Node\SNAP_V2\Workspaces\Workspace\drawings\SNAP Ver2 pack-n-go\Workgroups\NotInProject\CAPC1005X50L_C177.ipt
- C:\Users\Zara\Documents\hera-cad\Node\SNAP_V2\Workspaces\Workspace\drawings\SNAP Ver2 pack-n-go\Workgroups\NotInProject\CAPC1005X50L_C180.ipt
- C:\Users\Zara\Documents\hera-cad\Node\SNAP_V2\Workspaces\Workspace\drawings\SNAP Ver2 pack-n-go\Workgroups\NotInProject\CAPC1005X50L_C216.ipt
- C:\Users\Zara\Documents\hera-cad\Node\SNAP_V2\Workspaces\Workspace\drawings\SNAP Ver2 pack-n-go\Workgroups\NotInProject\CAPC1005X50L_C184.ipt
- C:\Users\Zara\Documents\hera-cad\Node\SNAP_V2\Workspaces\Workspace\drawings\SNAP Ver2 pack-n-go\Workgroups\NotInProject\CAPC1005X50L_C187.ipt
- C:\Users\Zara\Documents\hera-cad\Node\SNAP_V2\Workspaces\Workspace\drawings\SNAP Ver2 pack-n-go\Workgroups\NotInProject\CAPC1005X50L_C188.ipt
- C:\Users\Zara\Documents\hera-cad\Node\SNAP_V2\Workspaces\Workspace\drawings\SNAP Ver2 pack-n-go\Workgroups\NotInProject\CAPC1005X50L_C189.ipt
- C:\Users\Zara\Documents\hera-cad\Node\SNAP_V2\Workspaces\Workspace\drawings\SNAP Ver2 pack-n-go\Workgroups\NotInProject\CAPC1005X50L_C182.ipt
- C:\Users\Zara\Documents\hera-cad\Node\SNAP_V2\Workspaces\Workspace\drawings\SNAP Ver2 pack-n-go\Workgroups\NotInProject\CAPC1005X50L_C18.ipt
- C:\Users\Zara\Documents\hera-cad\Node\SNAP_V2\Workspaces\Workspace\drawings\SNAP Ver2 pack-n-go\Workgroups\NotInProject\CAPC1005X50L_C93.ipt
- C:\Users\Zara\Documents\hera-cad\Node\SNAP_V2\Workspaces\Workspace\drawings\SNAP Ver2 pack-n-go\Workgroups\NotInProject\CAPC1005X50L_C186.ipt
- C:\Users\Zara\Documents\hera-cad\Node\SNAP_V2\Workspaces\Workspace\drawings\SNAP Ver2 pack-n-go\Workgroups\NotInProject\CAPC1005X50L_C20.ipt
- C:\Users\Zara\Documents\hera-cad\Node\SNAP_V2\Workspaces\Workspace\drawings\SNAP Ver2 pack-n-go\Workgroups\NotInProject\CAPC1005X50L_C59.ipt
- C:\Users\Zara\Documents\hera-cad\Node\SNAP_V2\Workspaces\Workspace\drawings\SNAP Ver2 pack-n-go\Workgroups\NotInProject\CAPC1005X50L_C98.ipt
- C:\Users\Zara\Documents\hera-cad\Node\SNAP_V2\Workspaces\Workspace\drawings\SNAP Ver2 pack-n-go\Workgroups\NotInProject\CAPC1005X50L_C279.ipt
- C:\Users\Zara\Documents\hera-cad\Node\SNAP_V2\Workspaces\Workspace\drawings\SNAP Ver2 pack-n-go\Workgroups\NotInProject\CAPC1005X50L_C280.ipt
- C:\Users\Zara\Documents\hera-cad\Node\SNAP_V2\Workspaces\Workspace\drawings\SNAP Ver2 pack-n-go\Workgroups\NotInProject\CAPC1005X50L_C282.ipt
- C:\Users\Zara\Documents\hera-cad\Node\SNAP_V2\Workspaces\Workspace\drawings\SNAP Ver2 pack-n-go\Workgroups\NotInProject\CAPC1005X50L_C284.ipt
- C:\Users\Zara\Documents\hera-cad\Node\SNAP_V2\Workspaces\Workspace\drawings\SNAP Ver2 pack-n-go\Workgroups\NotInProject\CAPC1005X50L_C289.ipt
- C:\Users\Zara\Documents\hera-cad\Node\SNAP_V2\Workspaces\Workspace\drawings\SNAP Ver2 pack-n-go\Workgroups\NotInProject\CAPC1005X50L_C301.ipt
- C:\Users\Zara\Documents\hera-cad\Node\SNAP_V2\Workspaces\Workspace\drawings\SNAP Ver2 pack-n-go\Workgroups\NotInProject\CAPC1005X50L_C302.ipt
- C:\Users\Zara\Documents\hera-cad\Node\SNAP_V2\Workspaces\Workspace\drawings\SNAP Ver2 pack-n-go\Workgroups\NotInProject\CAPC1005X50L_C304.ipt
- C:\Users\Zara\Documents\hera-cad\Node\SNAP_V2\Workspaces\Workspace\drawings\SNAP Ver2 pack-n-go\Workgroups\NotInProject\CAPC1005X50L_C306.ipt
- C:\Users\Zara\Documents\hera-cad\Node\SNAP_V2\Workspaces\Workspace\drawings\SNAP Ver2 pack-n-go\Workgroups\NotInProject\CAPC1005X50L_C311.ipt
- C:\Users\Zara\Documents\hera-cad\Node\SNAP_V2\Workspaces\Workspace\drawings\SNAP Ver2 pack-n-go\Workgroups\NotInProject\CAPC1005X50L_C287.ipt
- C:\Users\Zara\Documents\hera-cad\Node\SNAP_V2\Workspaces\Workspace\drawings\SNAP Ver2 pack-n-go\Workgroups\NotInProject\CAPC1005X50L_C309.ipt
- C:\Users\Zara\Documents\hera-cad\Node\SNAP_V2\Workspaces\Workspace\drawings\SNAP Ver2 pack-n-go\Workgroups\NotInProject\CAPC1005X50L_C3.ipt
- C:\Users\Zara\Documents\hera-cad\Node\SNAP_V2\Workspaces\Workspace\drawings\SNAP Ver2 pack-n-go\Workgroups\NotInProject\CAPC1005X50L_C42.ipt
- C:\Users\Zara\Documents\hera-cad\Node\SNAP_V2\Workspaces\Workspace\drawings\SNAP Ver2 pack-n-go\Workgroups\NotInProject\CAPC1005X50L_C81.ipt
- C:\Users\Zara\Documents\hera-cad\Node\SNAP_V2\Workspaces\Workspace\drawings\SNAP Ver2 pack-n-go\Workgroups\NotInProject\CAPC1005X50L_C45.ipt
- C:\Users\Zara\Documents\hera-cad\Node\SNAP_V2\Workspaces\Workspace\drawings\SNAP Ver2 pack-n-go\Workgroups\NotInProject\CAPC1005X50L_C6.ipt
- C:\Users\Zara\Documents\hera-cad\Node\SNAP_V2\Workspaces\Workspace\drawings\SNAP Ver2 pack-n-go\Workgroups\NotInProject\CAPC1005X50L_C84.ipt
- C:\Users\Zara\Documents\hera-cad\Node\SNAP_V2\Workspaces\Workspace\drawings\SNAP Ver2 pack-n-go\Workgroups\NotInProject\CAPC1005X50L_C12.ipt
- C:\Users\Zara\Documents\hera-cad\Node\SNAP_V2\Workspaces\Workspace\drawings\SNAP Ver2 pack-n-go\Workgroups\NotInProject\CAPC1005X50L_C181.ipt
- C:\Users\Zara\Documents\hera-cad\Node\SNAP_V2\Workspaces\Workspace\drawings\SNAP Ver2 pack-n-go\Workgroups\NotInProject\CAPC1005X50L_C139.ipt
- C:\Users\Zara\Documents\hera-cad\Node\SNAP_V2\Workspaces\Workspace\drawings\SNAP Ver2 pack-n-go\Workgroups\NotInProject\CAPC1005X50L_C76.ipt
- C:\Users\Zara\Documents\hera-cad\Node\SNAP_V2\Workspaces\Workspace\drawings\SNAP Ver2 pack-n-go\Workgroups\NotInProject\CAPC1005X50L_C37.ipt
- C:\Users\Zara\Documents\hera-cad\Node\SNAP_V2\Workspaces\Workspace\drawings\SNAP Ver2 pack-n-go\Workgroups\NotInProject\CAPC1005X50L_C115.ipt
- C:\Users\Zara\Documents\hera-cad\Node\SNAP_V2\Workspaces\Workspace\drawings\SNAP Ver2 pack-n-go\Workgroups\NotInProject\CAPC1005X50L_C75.ipt
- C:\Users\Zara\Documents\hera-cad\Node\SNAP_V2\Workspaces\Workspace\drawings\SNAP Ver2 pack-n-go\Workgroups\NotInProject\CAPC1005X50L_C36.ipt
- C:\Users\Zara\Documents\hera-cad\Node\SNAP_V2\Workspaces\Workspace\drawings\SNAP Ver2 pack-n-go\Workgroups\NotInProject\CAPC1005X50L_C114.ipt
- C:\Users\Zara\Documents\hera-cad\Node\SNAP_V2\Workspaces\Workspace\drawings\SNAP Ver2 pack-n-go\Workgroups\NotInProject\CAPC1005X50L_C74.ipt
- C:\Users\Zara\Documents\hera-cad\Node\SNAP_V2\Workspaces\Workspace\drawings\SNAP Ver2 pack-n-go\Workgroups\NotInProject\CAPC1005X50L_C136.ipt
- C:\Users\Zara\Documents\hera-cad\Node\SNAP_V2\Workspaces\Workspace\drawings\SNAP Ver2 pack-n-go\Workgroups\NotInProject\CAPC1005X50L_C183.ipt
- C:\Users\Zara\Documents\hera-cad\Node\SNAP_V2\Workspaces\Workspace\drawings\SNAP Ver2 pack-n-go\Workgroups\NotInProject\CAPC1005X50L_C35.ipt
- C:\Users\Zara\Documents\hera-cad\Node\SNAP_V2\Workspaces\Workspace\drawings\SNAP Ver2 pack-n-go\Workgroups\NotInProject\CAPC1005X50L_C113.ipt
- C:\Users\Zara\Documents\hera-cad\Node\SNAP_V2\Workspaces\Workspace\drawings\SNAP Ver2 pack-n-go\Workgroups\NotInProject\CAPC1005X50L_C175.ipt
- C:\Users\Zara\Documents\hera-cad\Node\SNAP_V2\Workspaces\Workspace\drawings\SNAP Ver2 pack-n-go\Workgroups\NotInProject\CAPC1005X50L_C174.ipt
- C:\Users\Zara\Documents\hera-cad\Node\SNAP_V2\Workspaces\Workspace\drawings\SNAP Ver2 pack-n-go\Workgroups\NotInProject\CAPC1005X50L_C171.ipt
- C:\Users\Zara\Documents\hera-cad\Node\SNAP_V2\Workspaces\Workspace\drawings\SNAP Ver2 pack-n-go\Workgroups\NotInProject\CAPC1005X50L_C166.ipt
- C:\Users\Zara\Documents\hera-cad\Node\SNAP_V2\Workspaces\Workspace\drawings\SNAP Ver2 pack-n-go\Workgroups\NotInProject\CAPC1005X50L_C165.ipt
- C:\Users\Zara\Documents\hera-cad\Node\SNAP_V2\Workspaces\Workspace\drawings\SNAP Ver2 pack-n-go\Workgroups\NotInProject\CAPC1005X50L_C185.ipt
- C:\Users\Zara\Documents\hera-cad\Node\SNAP_V2\Workspaces\Workspace\drawings\SNAP Ver2 pack-n-go\Workgroups\NotInProject\CAPC1005X50L_C163.ipt
- C:\Users\Zara\Documents\hera-cad\Node\SNAP_V2\Workspaces\Workspace\drawings\SNAP Ver2 pack-n-go\Workgroups\NotInProject\CAPC1005X50L_C72.ipt
- C:\Users\Zara\Documents\hera-cad\Node\SNAP_V2\Workspaces\Workspace\drawings\SNAP Ver2 pack-n-go\Workgroups\NotInProject\CAPC1005X50L_C135.ipt
- C:\Users\Zara\Documents\hera-cad\Node\SNAP_V2\Workspaces\Workspace\drawings\SNAP Ver2 pack-n-go\Workgroups\NotInProject\CAPC1005X50L_C131.ipt
- C:\Users\Zara\Documents\hera-cad\Node\SNAP_V2\Workspaces\Workspace\drawings\SNAP Ver2 pack-n-go\Workgroups\NotInProject\CAPC1005X50L_C129.ipt
- C:\Users\Zara\Documents\hera-cad\Node\SNAP_V2\Workspaces\Workspace\drawings\SNAP Ver2 pack-n-go\Workgroups\NotInProject\CAPC1005X50L_C127.ipt
- C:\Users\Zara\Documents\hera-cad\Node\SNAP_V2\Workspaces\Workspace\drawings\SNAP Ver2 pack-n-go\Workgroups\NotInProject\CAPC1005X50L_C123.ipt
- C:\Users\Zara\Documents\hera-cad\Node\SNAP_V2\Workspaces\Workspace\drawings\SNAP Ver2 pack-n-go\Workgroups\NotInProject\CAPC1005X50L_C33.ipt
- C:\Users\Zara\Documents\hera-cad\Node\SNAP_V2\Workspaces\Workspace\drawings\SNAP Ver2 pack-n-go\Workgroups\NotInProject\CAPC1005X50L_C111.ipt
- C:\Users\Zara\Documents\hera-cad\Node\SNAP_V2\Workspaces\Workspace\drawings\SNAP Ver2 pack-n-go\Workgroups\NotInProject\CAPC1005X50L_C89.ipt
- C:\Users\Zara\Documents\hera-cad\Node\SNAP_V2\Workspaces\Workspace\drawings\SNAP Ver2 pack-n-go\Workgroups\NotInProject\CAPC1005X50L_C50.ipt
- C:\Users\Zara\Documents\hera-cad\Node\SNAP_V2\Workspaces\Workspace\drawings\SNAP Ver2 pack-n-go\Workgroups\NotInProject\CAPC1005X50L_C11.ipt
- C:\Users\Zara\Documents\hera-cad\Node\SNAP_V2\Workspaces\Workspace\drawings\SNAP Ver2 pack-n-go\Workgroups\NotInProject\CAPC1005X50L_C70.ipt
- C:\Users\Zara\Documents\hera-cad\Node\SNAP_V2\Workspaces\Workspace\drawings\SNAP Ver2 pack-n-go\Workgroups\NotInProject\CAPC1005X50L_C31.ipt
- C:\Users\Zara\Documents\hera-cad\Node\SNAP_V2\Workspaces\Workspace\drawings\SNAP Ver2 pack-n-go\Workgroups\NotInProject\CAPC1005X50L_C109.ipt
- C:\Users\Zara\Documents\hera-cad\Node\SNAP_V2\Workspaces\Workspace\drawings\SNAP Ver2 pack-n-go\Workgroups\NotInProject\CAPC1005X50L_C69.ipt
- C:\Users\Zara\Documents\hera-cad\Node\SNAP_V2\Workspaces\Workspace\drawings\SNAP Ver2 pack-n-go\Workgroups\NotInProject\CAPC1005X50L_C30.ipt
- C:\Users\Zara\Documents\hera-cad\Node\SNAP_V2\Workspaces\Workspace\drawings\SNAP Ver2 pack-n-go\Workgroups\NotInProject\CAPC1005X50L_C121.ipt
- C:\Users\Zara\Documents\hera-cad\Node\SNAP_V2\Workspaces\Workspace\drawings\SNAP Ver2 pack-n-go\Workgroups\NotInProject\CAPC1005X50L_C119.ipt
- C:\Users\Zara\Documents\hera-cad\Node\SNAP_V2\Workspaces\Workspace\drawings\SNAP Ver2 pack-n-go\Workgroups\NotInProject\CAPC1005X50L_C108.ipt
- C:\Users\Zara\Documents\hera-cad\Node\SNAP_V2\Workspaces\Workspace\drawings\SNAP Ver2 pack-n-go\Workgroups\NotInProject\CAPC1005X50L_C78.ipt
- C:\Users\Zara\Documents\hera-cad\Node\SNAP_V2\Workspaces\Workspace\drawings\SNAP Ver2 pack-n-go\Workgroups\NotInProject\CAPC1005X50L_C39.ipt
- C:\Users\Zara\Documents\hera-cad\Node\SNAP_V2\Workspaces\Workspace\drawings\SNAP Ver2 pack-n-go\Workgroups\NotInProject\CAPC1005X50L_C117.ipt
- C:\Users\Zara\Documents\hera-cad\Node\SNAP_V2\Workspaces\Workspace\drawings\SNAP Ver2 pack-n-go\Workgroups\NotInProject\CAPC1005X50L_C104.ipt
- C:\Users\Zara\Documents\hera-cad\Node\SNAP_V2\Workspaces\Workspace\drawings\SNAP Ver2 pack-n-go\Workgroups\NotInProject\CAPC1005X50L_C64.ipt
- C:\Users\Zara\Documents\hera-cad\Node\SNAP_V2\Workspaces\Workspace\drawings\SNAP Ver2 pack-n-go\Workgroups\NotInProject\CAPC1005X50L_C1.ipt
- C:\Users\Zara\Documents\hera-cad\Node\SNAP_V2\Workspaces\Workspace\drawings\SNAP Ver2 pack-n-go\Workgroups\NotInProject\CAPC1005X50L_C40.ipt
- C:\Users\Zara\Documents\hera-cad\Node\SNAP_V2\Workspaces\Workspace\drawings\SNAP Ver2 pack-n-go\Workgroups\NotInProject\CAPC1005X50L_C79.ipt
- C:\Users\Zara\Documents\hera-cad\Node\SNAP_V2\Workspaces\Workspace\drawings\SNAP Ver2 pack-n-go\Workgroups\NotInProject\CAPC1005X50L_C10.ipt
- C:\Users\Zara\Documents\hera-cad\Node\SNAP_V2\Workspaces\Workspace\drawings\SNAP Ver2 pack-n-go\Workgroups\NotInProject\CAPC1005X50L_C49.ipt
- C:\Users\Zara\Documents\hera-cad\Node\SNAP_V2\Workspaces\Workspace\drawings\SNAP Ver2 pack-n-go\Workgroups\NotInProject\CAPC1005X50L_C88.ipt
- C:\Users\Zara\Documents\hera-cad\Node\SNAP_V2\Workspaces\Workspace\drawings\SNAP Ver2 pack-n-go\Workgroups\NotInProject\CAPC1005X50L_C67.ipt
- C:\Users\Zara\Documents\hera-cad\Node\SNAP_V2\Workspaces\Workspace\drawings\SNAP Ver2 pack-n-go\Workgroups\NotInProject\CAPC1005X50L_C28.ipt
- C:\Users\Zara\Documents\hera-cad\Node\SNAP_V2\Workspaces\Workspace\drawings\SNAP Ver2 pack-n-go\Workgroups\NotInProject\CAPC1005X50L_C106.ipt
- C:\Users\Zara\Documents\hera-cad\Node\SNAP_V2\Workspaces\Workspace\drawings\SNAP Ver2 pack-n-go\Workgroups\NotInProject\CAPC1005X50L_C66.ipt
- C:\Users\Zara\Documents\hera-cad\Node\SNAP_V2\Workspaces\Workspace\drawings\SNAP Ver2 pack-n-go\Workgroups\NotInProject\CAPC1005X50L_C27.ipt
- C:\Users\Zara\Documents\hera-cad\Node\SNAP_V2\Workspaces\Workspace\drawings\SNAP Ver2 pack-n-go\Workgroups\NotInProject\CAPC1005X50L_C105.ipt
- C:\Users\Zara\Documents\hera-cad\Node\SNAP_V2\Workspaces\Workspace\drawings\SNAP Ver2 pack-n-go\Workgroups\NotInProject\CAPC1005X50L_C65.ipt
- C:\Users\Zara\Documents\hera-cad\Node\SNAP_V2\Workspaces\Workspace\drawings\SNAP Ver2 pack-n-go\Workgroups\NotInProject\CAPC1005X50L_C26.ipt
- C:\Users\Zara\Documents\hera-cad\Node\SNAP_V2\Workspaces\Workspace\drawings\SNAP Ver2 pack-n-go\Workgroups\NotInProject\CAPC1005X50L_C25.ipt
- C:\Users\Zara\Documents\hera-cad\Node\SNAP_V2\Workspaces\Workspace\drawings\SNAP Ver2 pack-n-go\Workgroups\NotInProject\CAPC1005X50L_C102.ipt
- C:\Users\Zara\Documents\hera-cad\Node\SNAP_V2\Workspaces\Workspace\drawings\SNAP Ver2 pack-n-go\Workgroups\NotInProject\CAPC1005X50L_C103.ipt
- C:\Users\Zara\Documents\hera-cad\Node\SNAP_V2\Workspaces\Workspace\drawings\SNAP Ver2 pack-n-go\Workgroups\NotInProject\CAPC1005X50L_C63.ipt
- C:\Users\Zara\Documents\hera-cad\Node\SNAP_V2\Workspaces\Workspace\drawings\SNAP Ver2 pack-n-go\Workgroups\NotInProject\CAPC1005X50L_C24.ipt
- C:\Users\Zara\Documents\hera-cad\Node\SNAP_V2\Workspaces\Workspace\drawings\SNAP Ver2 pack-n-go\Workgroups\NotInProject\CAPC1005X50L_C61.ipt
- C:\Users\Zara\Documents\hera-cad\Node\SNAP_V2\Workspaces\Workspace\drawings\SNAP Ver2 pack-n-go\Workgroups\NotInProject\CAPC1005X50L_C100.ipt
- C:\Users\Zara\Documents\hera-cad\Node\SNAP_V2\Workspaces\Workspace\drawings\SNAP Ver2 pack-n-go\Workgroups\NotInProject\CAPC1005X50L_C22.ipt
- C:\Users\Zara\Documents\hera-cad\Node\SNAP_V2\Workspaces\Workspace\drawings\SNAP Ver2 pack-n-go\Workgroups\NotInProject\CAPC1005X50L_C601.ipt
- C:\Users\Zara\Documents\hera-cad\Node\SNAP_V2\Workspaces\Workspace\drawings\SNAP Ver2 pack-n-go\Workgroups\NotInProject\CAPC1005X50L_C602.ipt
- C:\Users\Zara\Documents\hera-cad\Node\SNAP_V2\Workspaces\Workspace\drawings\SNAP Ver2 pack-n-go\Workgroups\NotInProject\CAPC1608X90N_C120.ipt
- C:\Users\Zara\Documents\hera-cad\Node\SNAP_V2\Workspaces\Workspace\drawings\SNAP Ver2 pack-n-go\Workgroups\NotInProject\CAPC1608X90N_C124.ipt
- C:\Users\Zara\Documents\hera-cad\Node\SNAP_V2\Workspaces\Workspace\drawings\SNAP Ver2 pack-n-go\Workgroups\NotInProject\CAPC1608X90N_C128.ipt
- C:\Users\Zara\Documents\hera-cad\Node\SNAP_V2\Workspaces\Workspace\drawings\SNAP Ver2 pack-n-go\Workgroups\NotInProject\CAPC1608X90N_C132.ipt
- C:\Users\Zara\Documents\hera-cad\Node\SNAP_V2\Workspaces\Workspace\drawings\SNAP Ver2 pack-n-go\Workgroups\NotInProject\CAPC1608X90N_C179.ipt
- C:\Users\Zara\Documents\hera-cad\Node\SNAP_V2\Workspaces\Workspace\drawings\SNAP Ver2 pack-n-go\Workgroups\NotInProject\CAPC1608X90N_C150.ipt